# Autodesk Inventor assembly: lower arm with pulley
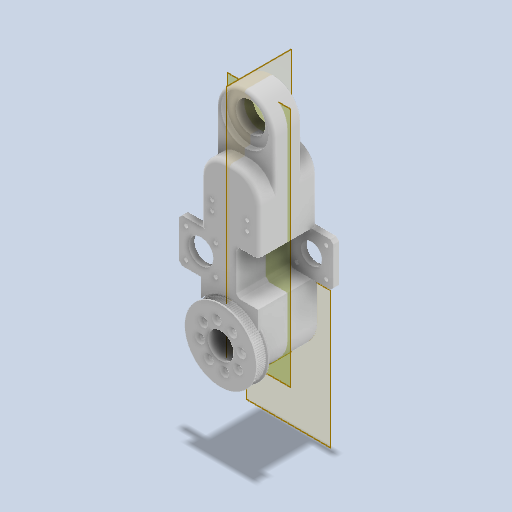
[picture p0: Inventor's stored thumbnail of the model, 512x512]
Saved by Autodesk Inventor 2024 (Build 280153000, 153)
## iProperties
Created: 2024-02-21
Part Number: lower arm with pulley
Document SubType Name: Assembly
Designer: MaartenGeorgesBuelen
Author: MaartenGeorgesBuelen
## Documents named in this file (3)
- C:\Users\MaartenGeorgesBuelen\Documents\Inventor\robot arm\arms\lower arm with pulley.iam
- C:\Users\MaartenGeorgesBuelen\Documents\Inventor\robot arm\arms\lower arm.ipt
- C:\Users\MaartenGeorgesBuelen\Documents\Inventor\robot arm\arms\lower arm pulley.ipt
## Components (2 placed, 2 different names)
1. lower arm:1 — Mate:2, Mate:3
2. lower arm pulley:1 — Mate:2, Mate:3
## Relationships (2: Mate 2)
- Mate:2: lower arm:1 ↔ lower arm pulley:1
- Mate:3: lower arm:1 ↔ lower arm pulley:1
